# Autodesk Inventor assembly: Cluth
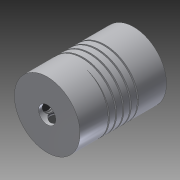
[picture p0: Inventor's stored thumbnail of the model, 180x180]
Saved by Autodesk Inventor 2014 SP1 (Build 180222100, 222)
## iProperties
Created: 2017-07-09
Part Number: Cluth
Document SubType Name: Assembly
Designer: Stepan
Author: Stepan
## Documents named in this file (3)
- D:\3DPrinter\Cluth\Cluth.iam
- D:\3DPrinter\Cluth\Bolt.ipt
- D:\3DPrinter\Cluth\Clutch.ipt
## Components (5 placed, 2 different names)
1. Bolt:1 — Жесткий:3
2. Bolt:2 — Жесткий:2
3. Bolt:3 — Жесткий:1
4. Bolt:4 — Жесткий:4
5. Clutch:1 — Жесткий:1, Жесткий:2, Жесткий:3, Жесткий:4
## Relationships (4: WeldJoint 4)
- Жесткий:1 [WeldJoint] (-0.25 mm): Bolt:3 ↔ Clutch:1
- Жесткий:2 [WeldJoint] (3.25 mm): Bolt:2 ↔ Clutch:1
- Жесткий:3 [WeldJoint] (0.25 mm): Bolt:1 ↔ Clutch:1
- Жесткий:4 [WeldJoint]: Bolt:4 ↔ Clutch:1
